# Autodesk Inventor assembly: Assembly proto panel
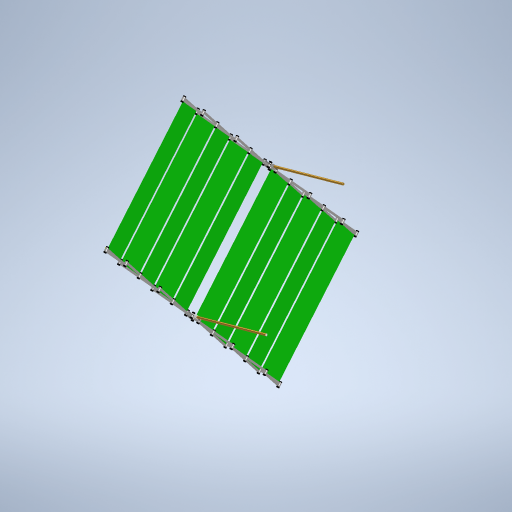
[picture p0: Inventor's stored thumbnail of the model, 512x512]
Saved by Autodesk Inventor 2024 (Build 280153000, 153)
## iProperties
Created: 2023-11-10
Part Number: Assembly proto panel
Document SubType Name: Assembly
Designer: chris
Author: chris
## Documents named in this file (8)
- C:\Users\chris\Desktop\στοιχεια 3\rover\Assembly proto panel.iam
- C:\Users\chris\Desktop\στοιχεια 3\rover\syndesh akrh.ipt
- C:\Users\chris\Desktop\στοιχεια 3\rover\atermonas.ipt
- C:\Users\chris\Desktop\στοιχεια 3\rover\syndesh panw.ipt
- C:\Users\chris\Desktop\στοιχεια 3\rover\phros.ipt
- C:\Users\chris\Desktop\στοιχεια 3\rover\vraxionas.ipt
- C:\Users\chris\Desktop\στοιχεια 3\rover\kinoymenh.ipt
- C:\Users\chris\Desktop\στοιχεια 3\rover\Panel.ipt
## Components (76 placed, 7 different names)
1. atermonas:1 — Mate:58, Mate:59, Mate:67
2. syndesh panw:1 — Mate:13, Mate:14, Mate:15, Mate:49, Mate:50, Mate:51, Mate:58, Mate:59, Mate:207
3. phros:1 — Mate:1, Mate:2, Mate:90
4. vraxionas:1 — Mate:1, Mate:2, Mate:3, Mate:4, Mate:5, Mate:6, Mate:91, Mate:122, Mate:123
5. phros:2 — Mate:3, Mate:4, Mate:7, Mate:8, Tangent:5, Tangent:6
6. phros:3 — Mate:9, Mate:14, Mate:15
7. phros:4 — Mate:10, Mate:12, Mate:93
8. phros:9 — Mate:5, Mate:6, Mate:70
9. vraxionas:2 — Mate:7, Mate:8, Mate:9, Mate:10, Mate:12, Mate:13, Mate:92, Mate:120, Mate:121
10. phros:19 — Mate:50, Mate:51
11. vraxionas:7 — Mate:65, Mate:66, Mate:80, Mate:81, Mate:116, Mate:117
12. phros:23 — Tangent:3, Tangent:4
13. vraxionas:8 — Mate:49, Mate:78, Mate:79, Mate:118, Mate:119
14. phros:24 — Mate:65, Mate:66, Mate:69
15. kinoymenh:1 — Mate:67, Mate:69, Mate:70, Mate:207
16. phros:25 — Mate:80, Mate:81
17. vraxionas:9 — Mate:79, Mate:94, Mate:104, Mate:112, Mate:113
18. phros:26 — Tangent:1, Tangent:2
19. vraxionas:10 — Mate:95, Mate:106, Mate:107, Mate:114, Mate:115
20. phros:27 — Mate:78
21. phros:28 — Mate:96, Mate:97, Tangent:9
22. vraxionas:11 — Mate:92, Mate:93, Mate:126, Mate:127
23. phros:29 — Tangent:7, Tangent:8
24. phros:30 — Mate:98
25. vraxionas:12 — Mate:90, Mate:91, Mate:99, Mate:124, Mate:125
26. phros:31 — Mate:94, Mate:103, Mate:110, Tangent:10
27. phros:32 — Mate:95, Mate:105, Mate:107
28. syndesh akrh:1 — Mate:98, Mate:99, Mate:101
29. syndesh akrh:2 — Mate:96, Mate:97, Mate:100, Mate:102, Mate:130, Mate:131
30. syndesh akrh:3 — Mate:105, Mate:106, Mate:109, Mate:111
31. syndesh akrh:4 — Mate:103, Mate:104, Mate:108, Mate:110, Mate:128, Mate:129
32. phros:33 — Mate:100, Mate:101, Mate:102
33. phros:34 — Mate:108, Mate:109, Mate:111
34. Panel:1 — Mate:112, Mate:113, Tangent:1
35. Panel:2 — Mate:114, Mate:115, Tangent:2
36. Panel:3 — Mate:118, Mate:119, Tangent:3, Mate:205, Mate:206, Tangent:11
37. Panel:6 — Mate:124, Mate:125, Tangent:7
38. Panel:7 — Mate:126, Mate:127, Tangent:8
39. Panel:9 — Mate:130, Mate:131, Tangent:9
40. Panel:10 — Mate:128, Mate:129, Tangent:10
41. Panel:11 — Mate:122, Mate:123, Tangent:6
42. Panel:12 — Mate:120, Mate:121, Tangent:5, Mate:203, Mate:204, Tangent:12
43. Panel:13 — Mate:116, Mate:117, Tangent:4
44. atermonas:2
45. syndesh panw:2
46. phros:35
47. vraxionas:13
48. phros:36 — Tangent:12
49. phros:37
50. phros:38
51. phros:39
52. vraxionas:14 — Mate:203, Mate:204
53. phros:40
54. vraxionas:15
55. phros:41 — Tangent:11
56. vraxionas:16 — Mate:205, Mate:206
57. phros:42
58. kinoymenh:2
59. phros:43
60. vraxionas:17
61. phros:44
62. vraxionas:18
63. phros:45
64. phros:46
65. vraxionas:19
66. phros:47
67. phros:48
68. vraxionas:20
69. phros:49
70. phros:50
71. syndesh akrh:5
72. syndesh akrh:6
73. syndesh akrh:7
74. syndesh akrh:8
75. phros:51
76. phros:52
## Relationships (183: Mate 166, Tangent 12, Angle 5)
- Mate:1: phros:1 ↔ vraxionas:1
- Mate:2: phros:1 ↔ vraxionas:1
- Mate:3: vraxionas:1 ↔ phros:2
- Mate:4: vraxionas:1 ↔ phros:2
- Mate:5: vraxionas:1 ↔ phros:9
- Mate:6: vraxionas:1 ↔ phros:9
- Mate:7: phros:2 ↔ vraxionas:2
- Mate:8: phros:2 ↔ vraxionas:2
- Mate:9: phros:3 ↔ vraxionas:2
- Mate:10: phros:4 ↔ vraxionas:2
- Mate:12: phros:4 ↔ vraxionas:2
- Mate:13: syndesh panw:1 ↔ vraxionas:2
- Mate:14: syndesh panw:1 ↔ phros:3
- Mate:15: syndesh panw:1 ↔ phros:3
- [Mate]: vraxionas:7 ↔ phros:23
- [Mate]: vraxionas:7 ↔ phros:23
- [Mate]: phros:23 ↔ vraxionas:8
- [Mate]: phros:23 ↔ vraxionas:8
- [Mate]: phros:19 ↔ vraxionas:8
- Mate:49: syndesh panw:1 ↔ vraxionas:8
- Mate:50: syndesh panw:1 ↔ phros:19
- Mate:51: syndesh panw:1 ↔ phros:19
- Mate:58: atermonas:1 ↔ syndesh panw:1
- Mate:59: atermonas:1 ↔ syndesh panw:1
- Mate:65: vraxionas:7 ↔ phros:24
- Mate:66: vraxionas:7 ↔ phros:24
- Mate:67: atermonas:1 ↔ kinoymenh:1
- Mate:69: phros:24 ↔ kinoymenh:1
- Mate:70: phros:9 ↔ kinoymenh:1
- [Mate]: vraxionas:9 ↔ phros:26
- [Mate]: vraxionas:9 ↔ phros:26
- [Mate]: phros:26 ↔ vraxionas:10
- [Mate]: phros:26 ↔ vraxionas:10
- [Mate]: phros:25 ↔ vraxionas:10
- [Mate]: vraxionas:9 ↔ phros:27
- [Mate]: vraxionas:9 ↔ phros:27
- Mate:78: vraxionas:8 ↔ phros:27
- Mate:79: vraxionas:8 ↔ vraxionas:9
- Mate:80: vraxionas:7 ↔ phros:25
- Mate:81: vraxionas:7 ↔ phros:25
- [Mate]: phros:28 ↔ vraxionas:11
- [Mate]: phros:28 ↔ vraxionas:11
- [Mate]: vraxionas:11 ↔ phros:29
- [Mate]: vraxionas:11 ↔ phros:29
- [Mate]: phros:29 ↔ vraxionas:12
- [Mate]: phros:29 ↔ vraxionas:12
- [Mate]: phros:30 ↔ vraxionas:12
- [Mate]: phros:30 ↔ vraxionas:12
- Mate:90: phros:1 ↔ vraxionas:12
- Mate:91: vraxionas:1 ↔ vraxionas:12
- Mate:92: vraxionas:2 ↔ vraxionas:11
- Mate:93: phros:4 ↔ vraxionas:11
- Mate:94: vraxionas:9 ↔ phros:31
- Mate:95: vraxionas:10 ↔ phros:32
- Mate:96: phros:28 ↔ syndesh akrh:2
- Mate:97: phros:28 ↔ syndesh akrh:2
- Mate:98: phros:30 ↔ syndesh akrh:1
- Mate:99: vraxionas:12 ↔ syndesh akrh:1
- Mate:100: syndesh akrh:2 ↔ phros:33
- Mate:101: syndesh akrh:1 ↔ phros:33
- Mate:102: syndesh akrh:2 ↔ phros:33
- Mate:103: phros:31 ↔ syndesh akrh:4
- Mate:104: vraxionas:9 ↔ syndesh akrh:4
- Mate:105: phros:32 ↔ syndesh akrh:3
- Mate:106: vraxionas:10 ↔ syndesh akrh:3
- Mate:107: vraxionas:10 ↔ phros:32
- Mate:108: syndesh akrh:4 ↔ phros:34
- Mate:109: syndesh akrh:3 ↔ phros:34
- Mate:110: phros:31 ↔ syndesh akrh:4
- Mate:111: syndesh akrh:3 ↔ phros:34
- Mate:112: vraxionas:9 ↔ Panel:1
- Mate:113: vraxionas:9 ↔ Panel:1
- Tangent:1: phros:26 ↔ Panel:1
- Mate:114: vraxionas:10 ↔ Panel:2
- Mate:115: vraxionas:10 ↔ Panel:2
- Tangent:2: phros:26 ↔ Panel:2
- Mate:116: vraxionas:7 ↔ Panel:13
- Mate:117: vraxionas:7 ↔ Panel:13
- Mate:118: vraxionas:8 ↔ Panel:3
- Mate:119: vraxionas:8 ↔ Panel:3
- Mate:120: vraxionas:2 ↔ Panel:12
- Mate:121: vraxionas:2 ↔ Panel:12
- Mate:122: vraxionas:1 ↔ Panel:11
- Mate:123: vraxionas:1 ↔ Panel:11
- Mate:124: vraxionas:12 ↔ Panel:6
- Mate:125: vraxionas:12 ↔ Panel:6
- Mate:126: vraxionas:11 ↔ Panel:7
- Mate:127: vraxionas:11 ↔ Panel:7
- Tangent:3: phros:23 ↔ Panel:3
- Tangent:4: phros:23 ↔ Panel:13
- Tangent:5: phros:2 ↔ Panel:12
- Tangent:6: phros:2 ↔ Panel:11
- Tangent:7: phros:29 ↔ Panel:6
- Tangent:8: phros:29 ↔ Panel:7
- Mate:128: syndesh akrh:4 ↔ Panel:10
- Mate:129: syndesh akrh:4 ↔ Panel:10
- Mate:130: syndesh akrh:2 ↔ Panel:9
- Mate:131: syndesh akrh:2 ↔ Panel:9
- Tangent:9: phros:28 ↔ Panel:9
- Tangent:10: phros:31 ↔ Panel:10
- [Mate]: phros:35 ↔ vraxionas:13
- [Mate]: phros:35 ↔ vraxionas:13
- [Mate]: vraxionas:13 ↔ phros:36
- [Mate]: vraxionas:13 ↔ phros:36
- [Mate]: vraxionas:13 ↔ phros:39
- [Mate]: vraxionas:13 ↔ phros:39
- [Mate]: phros:36 ↔ vraxionas:14
- [Mate]: phros:36 ↔ vraxionas:14
- [Mate]: phros:37 ↔ vraxionas:14
- [Mate]: phros:38 ↔ vraxionas:14
- [Mate]: phros:38 ↔ vraxionas:14
- [Mate]: syndesh panw:2 ↔ vraxionas:14
- [Mate]: syndesh panw:2 ↔ phros:37
- [Mate]: syndesh panw:2 ↔ phros:37
- [Mate]: vraxionas:15 ↔ phros:41
- [Mate]: vraxionas:15 ↔ phros:41
- [Mate]: phros:41 ↔ vraxionas:16
- [Mate]: phros:41 ↔ vraxionas:16
- [Mate]: phros:40 ↔ vraxionas:16
- [Mate]: syndesh panw:2 ↔ vraxionas:16
- [Mate]: syndesh panw:2 ↔ phros:40
- [Mate]: syndesh panw:2 ↔ phros:40
- [Mate]: atermonas:2 ↔ syndesh panw:2
- [Mate]: atermonas:2 ↔ syndesh panw:2
- [Mate]: vraxionas:15 ↔ phros:42
- [Mate]: vraxionas:15 ↔ phros:42
- [Mate]: atermonas:2 ↔ kinoymenh:2
- [Angle] (0 deg): syndesh panw:2 ↔ vraxionas:16
- [Mate]: syndesh panw:2 ↔ kinoymenh:2
- [Mate]: phros:42 ↔ kinoymenh:2
- [Mate]: phros:39 ↔ kinoymenh:2
- [Mate]: vraxionas:17 ↔ phros:44
- [Mate]: vraxionas:17 ↔ phros:44
- [Mate]: phros:44 ↔ vraxionas:18
- [Mate]: phros:44 ↔ vraxionas:18
- [Mate]: phros:43 ↔ vraxionas:18
- [Mate]: vraxionas:17 ↔ phros:45
- [Mate]: vraxionas:17 ↔ phros:45
- [Mate]: vraxionas:16 ↔ phros:45
- [Mate]: vraxionas:16 ↔ vraxionas:17
- [Mate]: vraxionas:15 ↔ phros:43
- [Mate]: vraxionas:15 ↔ phros:43
- [Mate]: phros:46 ↔ vraxionas:19
- [Mate]: phros:46 ↔ vraxionas:19
- [Mate]: vraxionas:19 ↔ phros:47
- [Mate]: vraxionas:19 ↔ phros:47
- [Mate]: phros:47 ↔ vraxionas:20
- [Mate]: phros:47 ↔ vraxionas:20
- [Mate]: phros:48 ↔ vraxionas:20
- [Mate]: phros:48 ↔ vraxionas:20
- [Mate]: phros:35 ↔ vraxionas:20
- [Mate]: vraxionas:13 ↔ vraxionas:20
- [Mate]: vraxionas:14 ↔ vraxionas:19
- [Mate]: phros:38 ↔ vraxionas:19
- [Mate]: vraxionas:17 ↔ phros:49
- [Mate]: vraxionas:18 ↔ phros:50
- [Mate]: phros:46 ↔ syndesh akrh:6
- [Mate]: phros:46 ↔ syndesh akrh:6
- [Mate]: phros:48 ↔ syndesh akrh:5
- [Mate]: vraxionas:20 ↔ syndesh akrh:5
- [Mate]: syndesh akrh:6 ↔ phros:51
- [Mate]: syndesh akrh:5 ↔ phros:51
- [Mate]: syndesh akrh:6 ↔ phros:51
- [Mate]: phros:49 ↔ syndesh akrh:8
- [Mate]: vraxionas:17 ↔ syndesh akrh:8
- [Mate]: phros:50 ↔ syndesh akrh:7
- [Mate]: vraxionas:18 ↔ syndesh akrh:7
- [Mate]: vraxionas:18 ↔ phros:50
- [Mate]: syndesh akrh:8 ↔ phros:52
- [Mate]: syndesh akrh:7 ↔ phros:52
- [Angle] (0 deg): vraxionas:19 ↔ vraxionas:20
- [Angle] (0 deg): vraxionas:13 ↔ vraxionas:14
- [Angle] (0 deg): vraxionas:15 ↔ vraxionas:16
- [Angle] (0 deg): vraxionas:17 ↔ vraxionas:18
- [Mate]: phros:49 ↔ syndesh akrh:8
- [Mate]: syndesh akrh:7 ↔ phros:52
- Mate:203: Panel:12 ↔ vraxionas:14
- Mate:204: Panel:12 ↔ vraxionas:14
- Mate:205: Panel:3 ↔ vraxionas:16
- Mate:206: Panel:3 ↔ vraxionas:16
- Tangent:11: Panel:3 ↔ phros:41
- Tangent:12: Panel:12 ↔ phros:36
- Mate:207 (450 mm): syndesh panw:1 ↔ kinoymenh:1
## Named parameters: d32_d26 = 0 mm, d44_d17_d2 = 0 mm, d45_d18_d3 = 0 mm, d46_d21_d6 = 0 mm, d47_d22_d7 = 0 mm, d93_d76 = 0 mm, d94_d77 = 0 mm, d95_d32_d26 = 0 mm, d96_d44_d17_d2 = 0 mm, d97_d45_d18_d3 = 0 mm, d98_d46_d21_d6 = 0 mm, d99_d47_d22_d7 = 0 mm, d104_d0 = 0 mm, d105_d1 = 0 mm, d106_d2 = 0 mm, d107_d3 = 0 mm, d108_d6 = 0 mm, d109_d7 = 0 mm, d110_d9 = 0 mm, d111_d11 = 0 mm, d202_d164 = 0 mm, d203_d165 = 0 mm, d204_d119 = 0 mm, d205_d120 = 0 mm, d206_d121 = 0 mm, d207_d122 = 0 mm, d208_d123 = 0 mm, d209_d124 = 0 mm, d210_d125 = 0 mm, d211_d126 = 0 mm, d212_d127 = 0 mm, d213_d128 = 0 mm, d214_d129 = 0 mm, d215_d130 = 0 mm, d216_d131 = 0 mm, d217_d135 = 0 deg, d218_d136 = 170 deg, d219_d137 = 10 deg, d220_d138 = 0 deg, d221_d139 = 170 deg, d222_d140 = 10 deg, d223_d141 = 0 deg, d224_d142 = 170 deg, d225_d143 = 10 deg, d226_d144 = 0 deg, d227_d145 = 170 deg, d228_d146 = 10 deg, d229_d77 = 0 mm, d230_d78 = 0 mm, d231_d85 = 0 deg, d232_d86 = 87 deg, d233_d87 = 5 deg, d234_d88 = 0 mm, d235_d89 = 450 mm, d236_d90 = 50 mm, d237_d91 = 0 mm, d238_d92 = 0 mm, d239_d93_d76 = 0 mm, d240_d94_d77 = 0 mm, d241_d95_d32_d26 = 0 mm, d242_d96_d44_d17_d2 = 0 mm, d243_d97_d45_d18_d3 = 0 mm, d244_d98_d46_d21_d6 = 0 mm, d245_d99_d47_d22_d7 = 0 mm, d246_d100 = 0 mm, d247_d101 = 0 mm, d248_d102 = 0 mm, d249_d103 = 0 mm, d250_d104_d0 = 0 mm, d251_d105_d1 = 0 mm, d252_d106_d2 = 0 mm, d253_d107_d3 = 0 mm, d254_d108_d6 = 0 mm, d255_d109_d7 = 0 mm, d256_d110_d9 = 0 mm, d257_d111_d11 = 0 mm, d258_d112 = 0 mm, d259_d113 = 0 mm, d260_d114 = 0 mm, d261_d115 = 0 mm, d262_d116 = 0 mm, d263_d117 = 0 mm, d264_d118 = 0 mm, d265_d5 = 0 mm, d266_d6 = 0 mm, d267_d7 = 0 mm, d268_d8 = 0 mm, d269_d9 = 0 mm, d270_d11 = 0 mm, d271_d12 = 0 mm, d272_d13 = 0 mm, d273_d14 = 0 mm, d274_d32_d26 = 0 mm, d275_d44_d17_d2 = 0 mm, d276_d45_d18_d3 = 0 mm, d277_d46_d21_d6 = 0 mm, d278_d47_d22_d7 = 0 mm, d279_d52 = 0 mm, d280_d53 = 0 mm, d281_d54 = 0 mm, d282_d61 = 0 mm, d283_d62 = 0 mm, d284_d76 = 0 mm, d285_d0 = 0 mm, d286_d1 = 0 mm, d287_d2 = 0 mm, d288_d3 = 0 mm, d289_d4 = 0 mm
